# Autodesk Inventor assembly: Gantry Corner Plate Assembly
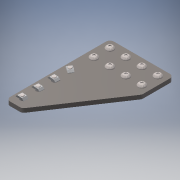
[picture p0: Inventor's stored thumbnail of the model, 180x180]
Saved by Autodesk Inventor 2017 (Build 210142000, 142)
## iProperties
Created: 2017-01-04
Part Number: Gantry Corner Plate Assembly
Document SubType Name: Assembly
Designer: Ali
Author: Ali
## Documents named in this file (3)
- C:\Users\Ali\Desktop\roboticFarm-master\Models2\Gantry\Ali\Gantry Corner Plate Assembly.iam
- C:\Users\Ali\Desktop\roboticFarm-master\Models2\Gantry\Ali\Gantry Corner Plate.ipt
- C:\Users\Ali\Desktop\roboticFarm-master\Models2\Gantry\Ali\M5 Screw with Tee Nut.iam
## Components (13 placed, 2 different names)
1. Gantry Corner Plate:1 — Rigid:1, Rigid:2, Rigid:3, Rigid:4, Rigid:5, Rigid:6, Rigid:7, Rigid:8, Rigid:10, Rigid:11, Rigid:12, Rigid:13
2. M5 Screw with Tee Nut:1 [sub-assembly] — Rigid:1
3. M5 Screw with Tee Nut:2 [sub-assembly] — Rigid:6
4. M5 Screw with Tee Nut:3 [sub-assembly] — Rigid:5
5. M5 Screw with Tee Nut:4 [sub-assembly] — Rigid:3
6. M5 Screw with Tee Nut:5 [sub-assembly] — Rigid:7
7. M5 Screw with Tee Nut:6 [sub-assembly] — Rigid:4
8. M5 Screw with Tee Nut:7 [sub-assembly] — Rigid:8
9. M5 Screw with Tee Nut:8 [sub-assembly] — Rigid:2
10. M5 Screw with Tee Nut:9 [sub-assembly] — Rigid:10
11. M5 Screw with Tee Nut:10 [sub-assembly] — Rigid:11
12. M5 Screw with Tee Nut:11 [sub-assembly] — Rigid:12
13. M5 Screw with Tee Nut:14 [sub-assembly] — Rigid:13
## Relationships (12: WeldJoint 12)
- Rigid:1 [WeldJoint]: Gantry Corner Plate:1 ↔ M5 Screw with Tee Nut:1
- Rigid:2 [WeldJoint]: Gantry Corner Plate:1 ↔ M5 Screw with Tee Nut:8
- Rigid:3 [WeldJoint]: Gantry Corner Plate:1 ↔ M5 Screw with Tee Nut:4
- Rigid:4 [WeldJoint]: Gantry Corner Plate:1 ↔ M5 Screw with Tee Nut:6
- Rigid:5 [WeldJoint]: Gantry Corner Plate:1 ↔ M5 Screw with Tee Nut:3
- Rigid:6 [WeldJoint]: Gantry Corner Plate:1 ↔ M5 Screw with Tee Nut:2
- Rigid:7 [WeldJoint]: Gantry Corner Plate:1 ↔ M5 Screw with Tee Nut:5
- Rigid:8 [WeldJoint]: Gantry Corner Plate:1 ↔ M5 Screw with Tee Nut:7
- Rigid:10 [WeldJoint]: Gantry Corner Plate:1 ↔ M5 Screw with Tee Nut:9
- Rigid:11 [WeldJoint]: Gantry Corner Plate:1 ↔ M5 Screw with Tee Nut:10
- Rigid:12 [WeldJoint]: Gantry Corner Plate:1 ↔ M5 Screw with Tee Nut:11
- Rigid:13 [WeldJoint]: Gantry Corner Plate:1 ↔ M5 Screw with Tee Nut:14
